# Autodesk Inventor assembly: tail_p3
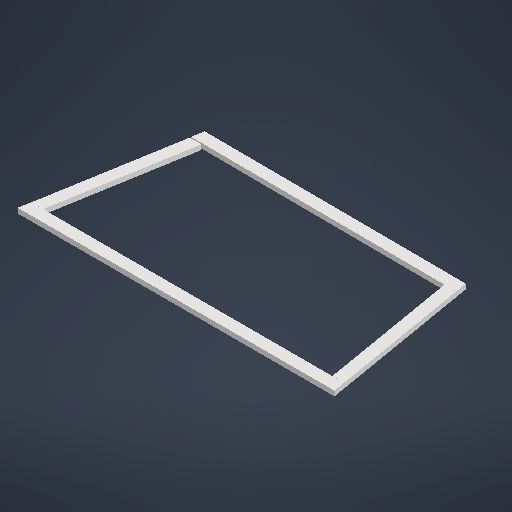
[picture p0: Inventor's stored thumbnail of the model, 512x512]
Saved by Autodesk Inventor 2027.1 (Build 311270010, 270A)
## iProperties
Created: 2026-09-01
Part Number: tail_p3
Document SubType Name: Assembly
Designer: jorda
Author: jorda
## Documents named in this file (4)
- C:\Users\jorda\OneDrive\Documents\GitHub\USC-ASME-TigerBurn-2026\CAD\Tail\tail_p3.iam
- C:\Users\jorda\OneDrive\Documents\GitHub\USC-ASME-TigerBurn-2026\CAD\Tail\S_2x4x48.76.ipt
- C:\Users\jorda\OneDrive\Documents\GitHub\USC-ASME-TigerBurn-2026\CAD\Tail\S_2x4x82.ipt
- C:\Users\jorda\OneDrive\Documents\GitHub\USC-ASME-TigerBurn-2026\CAD\Tail\S_2x4x96b.ipt
## Components (4 placed, 3 different names)
1. S_2x4x48.76:1 — Mate:10, Flush:9, Flush:10
2. S_2x4x96b:1 — Mate:10, Flush:9, Flush:10, Mate:11, Mate:12, Flush:11
3. S_2x4x48.76:2 — Mate:11, Mate:12, Flush:11, Flush:12, Flush:13, Mate:13
4. S_2x4x82:1 — Flush:12, Flush:13, Mate:13
## Relationships (9: Flush 5, Mate 4)
- Mate:10: S_2x4x48.76:1 ↔ S_2x4x96b:1
- Flush:9: S_2x4x48.76:1 ↔ S_2x4x96b:1
- Flush:10: S_2x4x48.76:1 ↔ S_2x4x96b:1
- Mate:11: S_2x4x96b:1 ↔ S_2x4x48.76:2
- Mate:12: S_2x4x96b:1 ↔ S_2x4x48.76:2
- Flush:11: S_2x4x96b:1 ↔ S_2x4x48.76:2
- Flush:12: S_2x4x48.76:2 ↔ S_2x4x82:1
- Flush:13: S_2x4x48.76:2 ↔ S_2x4x82:1
- Mate:13: S_2x4x48.76:2 ↔ S_2x4x82:1
